# Autodesk Inventor assembly: RightShoulderUnit
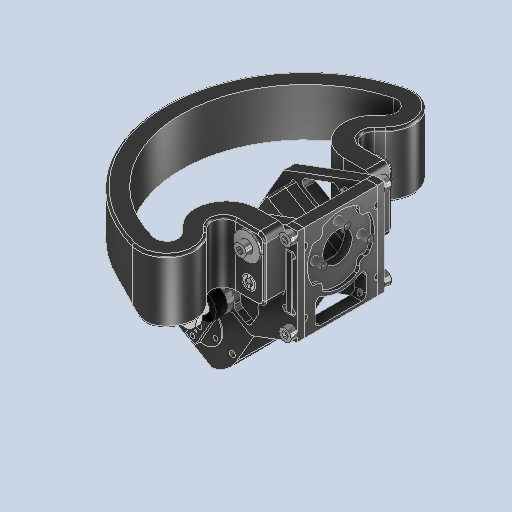
[picture p0: Inventor's stored thumbnail of the model, 512x512]
Saved by Autodesk Inventor 2024.2 (Build 282272000, 272)
## iProperties
Created: 2024-01-17
Part Number: RightShoulderUnit
Document SubType Name: Assembly
Designer: Masato Kubotera
Mass: 221.524 g
Surface Area: 458.526 cm^2
Volume: 116.896 cm^3
Density: 1.89505 g/cm^3
Author: Masato Kubotera
## Documents named in this file (17)
- C:\Users\masato\OneDrive - Chiba Institute of Technology\CIT Brains\RoboCup2024\Mechanic\SUSTAINA-OP2\NativeFiles\Boby\UpperLimb\Shoulders\RightShoulderUnit.iam
- C:\Users\masato\OneDrive - Chiba Institute of Technology\CIT Brains\RoboCup2024\Mechanic\SUSTAINA-OP2\NativeFiles\Boby\UpperLimb\Shoulders\ShoulderHormFrame.ipt
- C:\Users\masato\OneDrive - Chiba Institute of Technology\CIT Brains\RoboCup2024\Mechanic\SUSTAINA-OP2\NativeFiles\Boby\COTS\Actuators\PMX-SCR-5203HV.ipt
- C:\Users\masato\OneDrive - Chiba Institute of Technology\CIT Brains\RoboCup2024\Mechanic\SUSTAINA-OP2\NativeFiles\Boby\COTS\Screws\CapScrew\UC-0308.ipt
- C:\Users\masato\OneDrive - Chiba Institute of Technology\CIT Brains\RoboCup2024\Mechanic\SUSTAINA-OP2\NativeFiles\Boby\COTS\Screws\CapScrew\FC-2615EB.ipt
- C:\Users\masato\OneDrive - Chiba Institute of Technology\CIT Brains\RoboCup2024\Mechanic\SUSTAINA-OP2\NativeFiles\Boby\COTS\Screws\CapScrew\FC-2620EB.ipt
- C:\Users\masato\OneDrive - Chiba Institute of Technology\CIT Brains\RoboCup2024\Mechanic\SUSTAINA-OP2\NativeFiles\Boby\COTS\Washers\Resin\CC-0612-50B.ipt
- C:\Users\masato\OneDrive - Chiba Institute of Technology\CIT Brains\RoboCup2024\Mechanic\SUSTAINA-OP2\NativeFiles\Boby\COTS\Washers\Metal\UUW-0412-30H.ipt
- C:\Users\masato\OneDrive - Chiba Institute of Technology\CIT Brains\RoboCup2024\Mechanic\SUSTAINA-OP2\NativeFiles\Boby\COTS\Washers\Metal\UUW-0412-20H.ipt
- C:\Users\masato\OneDrive - Chiba Institute of Technology\CIT Brains\RoboCup2024\Mechanic\SUSTAINA-OP2\NativeFiles\Boby\COTS\Spacers\BRU-309S.ipt
- C:\Users\masato\OneDrive - Chiba Institute of Technology\CIT Brains\RoboCup2024\Mechanic\SUSTAINA-OP2\NativeFiles\Boby\COTS\Washers\Metal\UUW-0312-10H.ipt
- C:\Users\masato\OneDrive - Chiba Institute of Technology\CIT Brains\RoboCup2024\Mechanic\SUSTAINA-OP2\NativeFiles\Boby\COTS\Screws\CapScrew\UC-0306.ipt
- C:\Users\masato\OneDrive - Chiba Institute of Technology\CIT Brains\RoboCup2024\Mechanic\SUSTAINA-OP2\NativeFiles\Boby\UpperLimb\Shoulders\ShoulderBumper.ipt
- C:\Users\masato\OneDrive - Chiba Institute of Technology\CIT Brains\RoboCup2024\Mechanic\SUSTAINA-OP2\NativeFiles\Boby\UpperLimb\Shoulders\ShoulderHornSideFrame_MIR.ipt
- C:\Users\masato\OneDrive - Chiba Institute of Technology\CIT Brains\RoboCup2024\Mechanic\SUSTAINA-OP2\NativeFiles\Boby\UpperLimb\Shoulders\ShoulderIdlerSideFrame_MIR.ipt
- C:\Users\masato\OneDrive - Chiba Institute of Technology\CIT Brains\RoboCup2024\Mechanic\SUSTAINA-OP2\NativeFiles\Boby\COTS\Screws\ScrewsWithShoulder\DBSY4-10-6.ipt
- C:\Users\masato\OneDrive - Chiba Institute of Technology\CIT Brains\RoboCup2024\Mechanic\SUSTAINA-OP2\NativeFiles\Boby\COTS\Screws\ScrewsWithShoulder\DBSY4-5-5.ipt
## Components (27 placed, 16 different names)
1. ShoulderHornSideFrame_MIR:1 — Insert:1, Insert:2, Insert:13, Insert:14, Insert:30, Insert:31, Insert:19, Insert:5, Insert:15, Angle:6
2. ShoulderIdlerSideFrame_MIR:1 — Insert:3, Insert:4, Insert:11, Insert:12, Insert:28, Insert:29, Insert:24, Insert:27, Insert:17
3. ShoulderHormFrame:1 — Mate:1, Angle:1, Flush:3, Insert:1, Insert:2, Insert:3, Insert:4, Insert:7, Insert:8, Insert:9
4. ShoulderBumper:1 — Insert:40, Insert:41, Insert:42, Insert:43
5. PMX-SCR-5203HV:1 — Insert:5, Insert:27, Angle:6
6. UC-0306:1 — Insert:36
7. UC-0306:3 — Insert:38
8. UC-0308:1 — Insert:7
9. UC-0308:2 — Insert:8
10. UC-0308:3 — Insert:9
11. UC-0308:5 — Insert:11
12. UC-0308:6 — Insert:12
13. UC-0308:7 — Insert:13
14. UC-0308:8 — Insert:14
15. FC-2615EB:1 — Insert:15
16. FC-2620EB:1 — Insert:17
17. UUW-0312-10H:1 — Insert:32, Insert:36
18. UUW-0312-10H:3 — Insert:34, Insert:38
19. UUW-0412-30H:1 — Insert:19, Insert:20, Insert:21
20. UUW-0412-20H:1 — Insert:24, Insert:25
21. CC-0612-50B:1 — Insert:20
22. BRU-309S:1 — Insert:28, Angle:5, Insert:32, Insert:40
23. BRU-309S:2 — Insert:29, Angle:2, Insert:41
24. BRU-309S:3 — Insert:30, Angle:3, Insert:34, Insert:42
25. BRU-309S:4 — Insert:31, Angle:4, Insert:43
26. DBSY4-10-6:1 — Insert:21
27. DBSY4-5-5:1 — Insert:25
## Relationships (40: Insert 32, Angle 6, Mate 1, Flush 1)
- Mate:1: ShoulderHormFrame:1
- Angle:1 (180 deg): ShoulderHormFrame:1
- Flush:3: ShoulderHormFrame:1
- Insert:1: ShoulderHornSideFrame_MIR:1 ↔ ShoulderHormFrame:1
- Insert:2: ShoulderHornSideFrame_MIR:1 ↔ ShoulderHormFrame:1
- Insert:3: ShoulderIdlerSideFrame_MIR:1 ↔ ShoulderHormFrame:1
- Insert:4: ShoulderIdlerSideFrame_MIR:1 ↔ ShoulderHormFrame:1
- Insert:5: ShoulderHornSideFrame_MIR:1 ↔ PMX-SCR-5203HV:1
- Insert:7: ShoulderHormFrame:1 ↔ UC-0308:1
- Insert:8: ShoulderHormFrame:1 ↔ UC-0308:2
- Insert:9: ShoulderHormFrame:1 ↔ UC-0308:3
- Insert:11: ShoulderIdlerSideFrame_MIR:1 ↔ UC-0308:5
- Insert:12: ShoulderIdlerSideFrame_MIR:1 ↔ UC-0308:6
- Insert:13: ShoulderHornSideFrame_MIR:1 ↔ UC-0308:7
- Insert:14: ShoulderHornSideFrame_MIR:1 ↔ UC-0308:8
- Insert:15: ShoulderHornSideFrame_MIR:1 ↔ FC-2615EB:1
- Insert:17: ShoulderIdlerSideFrame_MIR:1 ↔ FC-2620EB:1
- Insert:19: ShoulderHornSideFrame_MIR:1 ↔ UUW-0412-30H:1
- Insert:20: UUW-0412-30H:1 ↔ CC-0612-50B:1
- Insert:21: UUW-0412-30H:1 ↔ DBSY4-10-6:1
- Insert:24: ShoulderIdlerSideFrame_MIR:1 ↔ UUW-0412-20H:1
- Insert:25: UUW-0412-20H:1 ↔ DBSY4-5-5:1
- Insert:27: ShoulderIdlerSideFrame_MIR:1 ↔ PMX-SCR-5203HV:1
- Insert:28: ShoulderIdlerSideFrame_MIR:1 ↔ BRU-309S:1
- Insert:29: ShoulderIdlerSideFrame_MIR:1 ↔ BRU-309S:2
- Insert:30: ShoulderHornSideFrame_MIR:1 ↔ BRU-309S:3
- Insert:31: ShoulderHornSideFrame_MIR:1 ↔ BRU-309S:4
- Angle:2 (0 deg): BRU-309S:2
- Angle:3 (0 deg): BRU-309S:3
- Angle:4 (0 deg): BRU-309S:4
- Angle:5 (0 deg): BRU-309S:1
- Insert:32: UUW-0312-10H:1 ↔ BRU-309S:1
- Insert:34: UUW-0312-10H:3 ↔ BRU-309S:3
- Insert:36: UC-0306:1 ↔ UUW-0312-10H:1
- Insert:38: UC-0306:3 ↔ UUW-0312-10H:3
- Insert:40: ShoulderBumper:1 ↔ BRU-309S:1
- Insert:41: ShoulderBumper:1 ↔ BRU-309S:2
- Insert:42: ShoulderBumper:1 ↔ BRU-309S:3
- Insert:43: ShoulderBumper:1 ↔ BRU-309S:4
- Angle:6 (0 deg): ShoulderHornSideFrame_MIR:1 ↔ PMX-SCR-5203HV:1
